# Autodesk Inventor assembly: Magnet Mount
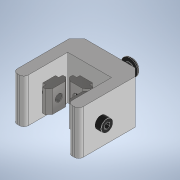
[picture p0: Inventor's stored thumbnail of the model, 180x180]
Saved by Autodesk Inventor 2022 (Build 260153000, 153)
## iProperties
Created: 2022-03-20
Part Number: Magnet Mount
Document SubType Name: Assembly
Designer: Nick
Author: Nick
## Documents named in this file (7)
- Y:\Projects\Bibble0\SubAsm\Magnet Mount.iam
- Y:\Projects\Bibble0\3D printed\Magnet Mount.ipt
- Y:\Projects\Bibble0\Hardware\10mm M4 Ball.ipt
- Y:\Projects\Bibble0\Hardware\Magnet.ipt
- Y:\Projects\Bibble0\Hardware\M3 x 8 mm SHCS.ipt
- Y:\Projects\Bibble0\Hardware\M3 T-Slot Nut.ipt
- Y:\Projects\Bibble0\Hardware\M4 x 8 mm BHCS.ipt
## Components (10 placed, 6 different names)
1. Magnet Mount:1 — Insert:1, Insert:2, Insert:3, Angle:1, Insert:5, Insert:6, Insert:7, Insert:8
2. 10mm M4 Ball:1 — Tangent:1, Mate:1, Mate:2, Insert:4
3. Magnet:1 — Insert:1, Tangent:1, Mate:1, Mate:2
4. M3 x 8 mm SHCS:1 — Insert:2
5. M3 T-Slot Nut:1 — Insert:3, Angle:1, Angle:2
6. M4 x 8 mm BHCS:1 — Insert:4
7. M3 x 8 mm SHCS:2 — Insert:5
8. M3 x 8 mm SHCS:3 — Insert:6
9. M3 T-Slot Nut:2 — Insert:8, Angle:2, Angle:3
10. M3 T-Slot Nut:3 — Insert:7, Angle:3
## Relationships (14: Insert 8, Angle 3, Mate 2, Tangent 1)
- Insert:1: Magnet Mount:1 ↔ Magnet:1
- Tangent:1: 10mm M4 Ball:1 ↔ Magnet:1
- Mate:1: 10mm M4 Ball:1 ↔ Magnet:1
- Mate:2: 10mm M4 Ball:1 ↔ Magnet:1
- Insert:2: Magnet Mount:1 ↔ M3 x 8 mm SHCS:1
- Insert:3 (1.5 mm): Magnet Mount:1 ↔ M3 T-Slot Nut:1
- Angle:1 (0 deg): Magnet Mount:1 ↔ M3 T-Slot Nut:1
- Insert:4 (1.5 mm): 10mm M4 Ball:1 ↔ M4 x 8 mm BHCS:1
- Insert:5: Magnet Mount:1 ↔ M3 x 8 mm SHCS:2
- Insert:6: Magnet Mount:1 ↔ M3 x 8 mm SHCS:3
- Insert:7 (1.5 mm): Magnet Mount:1 ↔ M3 T-Slot Nut:3
- Insert:8 (1.5 mm): Magnet Mount:1 ↔ M3 T-Slot Nut:2
- Angle:2 (0 deg): M3 T-Slot Nut:1 ↔ M3 T-Slot Nut:2
- Angle:3 (0 deg): M3 T-Slot Nut:2 ↔ M3 T-Slot Nut:3
